# Autodesk Inventor assembly: din_damper_connector_complete
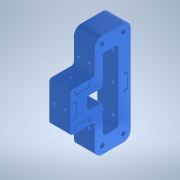
[picture p0: Inventor's stored thumbnail of the model, 180x180]
Saved by Autodesk Inventor 2021 (Build 250183000, 183)
## iProperties
Created: 2020-10-27
Part Number: din_damper_connector_complete
Document SubType Name: Assembly
Designer: Mateusz
Author: Mateusz
## Documents named in this file (3)
- D:\Projekty\UAV\CAD\din_connector_wheel.iam
- D:\Projekty\UAV\CAD\din_connector.ipt
- D:\Projekty\UAV\CAD\damping_system_housing_connector.ipt
## Components (3 placed, 2 different names)
1. din_connector:1 — Mate:1, Mate:2, Flush:1, Flush:3, Flush:4, Flush:5, Mate:7
2. damping_system_housing_connector:1 — Mate:1, Flush:4, Flush:5
3. damping_system_housing_connector:2 — Mate:2, Flush:1, Flush:3, Mate:8
## Relationships (8: Mate 4, Flush 4)
- Mate:1: din_connector:1 ↔ damping_system_housing_connector:1
- Mate:2: din_connector:1 ↔ damping_system_housing_connector:2
- Flush:1: din_connector:1 ↔ damping_system_housing_connector:2
- Flush:3: din_connector:1 ↔ damping_system_housing_connector:2
- Flush:4: din_connector:1 ↔ damping_system_housing_connector:1
- Flush:5: din_connector:1 ↔ damping_system_housing_connector:1
- Mate:7: din_connector:1
- Mate:8: damping_system_housing_connector:2
